# Autodesk Inventor assembly: robot-side-assembly
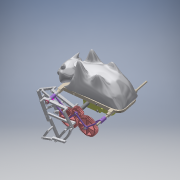
[picture p0: Inventor's stored thumbnail of the model, 180x180]
Saved by Autodesk Inventor 2017 (Build 210142000, 142)
## iProperties
Created: 2021-01-24
Part Number: robot-side-assembly
Document SubType Name: Assembly
Designer: agustin
Author: agustin
## Documents named in this file (42)
- D:\Agustin\Mis proyectos\Mechanisms\WalkingRobot\robot-side-assembly.iam
- D:\Agustin\Mis proyectos\Mechanisms\WalkingRobot\base-bone.ipt
- D:\Agustin\Mis proyectos\Mechanisms\WalkingRobot\bone0.ipt
- D:\Agustin\Mis proyectos\Mechanisms\WalkingRobot\bone1.ipt
- D:\Agustin\Mis proyectos\Mechanisms\WalkingRobot\bone2.ipt
- D:\Agustin\Mis proyectos\Mechanisms\WalkingRobot\bone3.ipt
- D:\Agustin\Mis proyectos\Mechanisms\WalkingRobot\bone4.ipt
- D:\Agustin\Mis proyectos\Mechanisms\WalkingRobot\bone5.ipt
- D:\Agustin\Mis proyectos\Mechanisms\WalkingRobot\toe1.ipt
- D:\Agustin\Mis proyectos\Mechanisms\WalkingRobot\toe2.ipt
- D:\Agustin\Mis proyectos\Mechanisms\WalkingRobot\bone6.ipt
- D:\Agustin\Mis proyectos\Mechanisms\WalkingRobot\bone7.ipt
- D:\Agustin\Mis proyectos\Mechanisms\WalkingRobot\chasis.ipt
- D:\Agustin\Mis proyectos\Mechanisms\WalkingRobot\DCMotor.ipt
- D:\Agustin\Mis proyectos\Mechanisms\WalkingRobot\battery-holder-robot.ipt
- D:\Agustin\Mis proyectos\Mechanisms\WalkingRobot\batter-holder.ipt
- D:\Agustin\Mis proyectos\Mechanisms\WalkingRobot\Servo.ipt
- D:\Agustin\Mis proyectos\Mechanisms\WalkingRobot\base-bone_MIR.ipt
- D:\Agustin\Mis proyectos\Mechanisms\WalkingRobot\bone0_MIR.ipt
- D:\Agustin\Mis proyectos\Mechanisms\WalkingRobot\bone1_MIR.ipt
- D:\Agustin\Mis proyectos\Mechanisms\WalkingRobot\bone2_MIR.ipt
- D:\Agustin\Mis proyectos\Mechanisms\WalkingRobot\bone3_MIR.ipt
- D:\Agustin\Mis proyectos\Mechanisms\WalkingRobot\bone4_MIR.ipt
- D:\Agustin\Mis proyectos\Mechanisms\WalkingRobot\bone5_MIR.ipt
- D:\Agustin\Mis proyectos\Mechanisms\WalkingRobot\toe1_MIR.ipt
- D:\Agustin\Mis proyectos\Mechanisms\WalkingRobot\toe2_MIR.ipt
- D:\Agustin\Mis proyectos\Mechanisms\WalkingRobot\bone6_MIR.ipt
- D:\Agustin\Mis proyectos\Mechanisms\WalkingRobot\bone7_MIR.ipt
- D:\Agustin\Mis proyectos\Mechanisms\WalkingRobot\gear1-shaft.ipt
- D:\Agustin\Mis proyectos\Mechanisms\WalkingRobot\gear-holder.ipt
- D:\Agustin\Mis proyectos\Mechanisms\WalkingRobot\small-gear.ipt
- D:\Agustin\Mis proyectos\Mechanisms\WalkingRobot\big-gear.ipt
- D:\Agustin\Mis proyectos\Mechanisms\WalkingRobot\gear2-shaft.ipt
- D:\Agustin\Mis proyectos\Mechanisms\WalkingRobot\dc-driver.ipt
- D:\Agustin\Mis proyectos\Mechanisms\WalkingRobot\node-mcu.ipt
- D:\Agustin\Mis proyectos\Mechanisms\WalkingRobot\ultrasound.ipt
- D:\Agustin\Mis proyectos\Mechanisms\WalkingRobot\head.ipt
- D:\Agustin\Mis proyectos\Mechanisms\WalkingRobot\shell.ipt
- D:\Agustin\Mis proyectos\Mechanisms\WalkingRobot\servo-shaft.ipt
- C:\Users\agustin\Documents\Inventor\Content Center Files\R2017\en-US\ANSI B18.3.4M(2)\ANSI B18.3.4M - M3 x 0.5 x 25(1).ipt
- C:\Users\agustin\Documents\Inventor\Content Center Files\R2017\en-US\AS 1112 (4)\AS 1112 - M3(2).ipt
- D:\Agustin\Mis proyectos\Mechanisms\WalkingRobot\washer.ipt
## Components (51 placed, 41 different names)
1. base-bone:1 — Mate:1, Mate:2, Mate:3, Mate:5, Mate:13, Mate:15, Mate:17, Mate:18
2. bone0:1 — Mate:5, Mate:6, Mate:22, Mate:25, Mate:152, Mate:154, Mate:194
3. bone1:1 — Mate:3, Mate:4, Mate:11, Mate:17, Mate:19, Mate:20
4. bone2:1 — Mate:2, Mate:12, Mate:18
5. bone3:1 — Mate:10, Mate:11, Mate:12, Mate:20
6. bone4:1 — Mate:4, Mate:7, Mate:8, Mate:19, Mate:23
7. bone5:1 — Mate:6, Mate:7, Mate:14, Mate:21, Mate:22
8. toe1:1 — Mate:8, Mate:9, Mate:23, Mate:24
9. toe2:1 — Mate:9, Mate:10, Mate:24
10. bone6:1 — Mate:1, Mate:16, Mate:153, Angle:3, Mate:156
11. bone7:1 — Mate:13, Mate:14, Mate:15, Mate:16, Mate:21
12. chasis:1 — Mate:25, Mate:121, Mate:122, Mate:134, Mate:152, Angle:6, Angle:7, Angle:8, Mate:166, Mate:167, Mate:168, Mate:169, Mate:172, Mate:173, Mate:174, Mate:175, Mate:176, Mate:177, Mate:178, Angle:11, Flush:13, Flush:14, Mate:189, Mate:190, Mate:191, Angle:12, Mate:193
13. battery-holder-robot:1 — Mate:44, Mate:179, Mate:180, Angle:11, Flush:11, Flush:12, Mate:192
14. batter-holder:1 — Mate:44, Mate:192
15. Servo:1 — Mate:163, Mate:164, Mate:191, Angle:12
16. base-bone_MIR:1 — Mate:49, Mate:50, Mate:51, Mate:52, Mate:53, Mate:67, Mate:70, Mate:72
17. bone0_MIR:1 — Mate:49, Mate:59, Mate:61, Mate:121, Mate:122
18. bone1_MIR:1 — Mate:50, Mate:51, Mate:54, Mate:56, Mate:57, Mate:58
19. bone2_MIR:1 — Mate:52, Mate:53, Mate:55
20. bone3_MIR:1 — Mate:54, Mate:55, Mate:56, Mate:65
21. bone4_MIR:1 — Mate:57, Mate:58, Mate:60, Mate:62, Mate:63
22. bone5_MIR:1 — Mate:59, Mate:60, Mate:61, Mate:68, Mate:71
23. toe1_MIR:1 — Mate:62, Mate:63, Mate:64, Mate:66
24. toe2_MIR:1 — Mate:64, Mate:65, Mate:66
25. bone6_MIR:1 — Mate:67, Mate:69, Mate:146, Angle:3
26. bone7_MIR:1 — Mate:68, Mate:69, Mate:70, Mate:71, Mate:72
27. gear1-shaft:1 — Mate:135, Mate:138, Mate:151, Angle:5, Mate:170, Mate:171
28. gear-holder:1 — Mate:134, Mate:135, Mate:136, Mate:137, Mate:144, Mate:146, Mate:147, Mate:151
29. gear-holder:2 — Mate:136, Mate:137, Mate:139, Mate:140, Mate:147, Mate:153, Mate:154
30. Spur Gear2:1 — Mate:138, Flush:5, Flush:6, Mate:144, Rotation:1, Angle:5, Rotation:2
31. Spur Gear1:1 — Mate:139, Flush:6, Mate:142, Flush:8, Mate:155, Rotation:1
32. Spur Gear1:2 — Mate:140, Flush:5, Mate:141, Mate:143, Flush:7, Rotation:2
33. gear2-shaft:1 — Mate:141, Mate:143, Flush:7
34. gear2-shaft:2 — Mate:142, Flush:8, Mate:155, Mate:156
35. dc-driver:1 — Angle:6, Angle:9, Mate:189
36. node-mcu:1 — Angle:7, Angle:8, Angle:9, Mate:190
37. ultrasound:1 — Mate:161, Mate:162, Angle:10
38. head:1 — Mate:161, Mate:162, Angle:10, Mate:165, Flush:9, Flush:10
39. shell:1 — Mate:166
40. servo-shaft:1 — Mate:163, Mate:164, Mate:165, Flush:9, Flush:10
41. DCMotor:1 — Mate:167, Mate:168, Mate:169, Mate:170, Mate:171, Mate:181, Mate:182
42. DCMotor:2 — Mate:172, Mate:173, Mate:174, Mate:179, Mate:180, Mate:183, Mate:184
43. Forged Hexagon Socket Button Head Cap Screw - Metric M3 x 0.5 x 25:1 — Mate:176, Mate:177, Mate:188
44. Forged Hexagon Socket Button Head Cap Screw - Metric M3 x 0.5 x 25:2 — Mate:175, Mate:178, Mate:187
45. Forged Hexagon Socket Button Head Cap Screw - Metric M3 x 0.5 x 25:3 — Mate:181, Mate:182, Mate:186
46. Forged Hexagon Socket Button Head Cap Screw - Metric M3 x 0.5 x 25:4 — Mate:183, Mate:184, Mate:185
47. AS 1112 (4) - Metric M3:1 — Mate:185, Flush:12
48. AS 1112 (4) - Metric M3:2 — Mate:187, Flush:13
49. AS 1112 (4) - Metric M3:3 — Mate:188, Flush:14
50. AS 1112 (4) - Metric M3:4 — Mate:186, Flush:11
51. washer:1 — Mate:193, Mate:194
## Relationships (126: Mate 105, Flush 10, Angle 9, RelateRotation 2)
- Mate:1: base-bone:1 ↔ bone6:1
- Mate:2: base-bone:1 ↔ bone2:1
- Mate:3: base-bone:1 ↔ bone1:1
- Mate:4: bone1:1 ↔ bone4:1
- Mate:5: base-bone:1 ↔ bone0:1
- Mate:6: bone0:1 ↔ bone5:1
- Mate:7: bone4:1 ↔ bone5:1
- Mate:8: bone4:1 ↔ toe1:1
- Mate:9: toe1:1 ↔ toe2:1
- Mate:10: bone3:1 ↔ toe2:1
- Mate:11: bone1:1 ↔ bone3:1
- Mate:12: bone2:1 ↔ bone3:1
- Mate:13: base-bone:1 ↔ bone7:1
- Mate:14: bone5:1 ↔ bone7:1
- Mate:15: base-bone:1 ↔ bone7:1
- Mate:16: bone6:1 ↔ bone7:1
- Mate:17: base-bone:1 ↔ bone1:1
- Mate:18: base-bone:1 ↔ bone2:1
- Mate:19: bone1:1 ↔ bone4:1
- Mate:20: bone1:1 ↔ bone3:1
- Mate:21: bone5:1 ↔ bone7:1
- Mate:22: bone0:1 ↔ bone5:1
- Mate:23: bone4:1 ↔ toe1:1
- Mate:24: toe1:1 ↔ toe2:1
- Mate:25: bone0:1 ↔ chasis:1
- Mate:44: battery-holder-robot:1 ↔ batter-holder:1
- Mate:49: base-bone_MIR:1 ↔ bone0_MIR:1
- Mate:50: base-bone_MIR:1 ↔ bone1_MIR:1
- Mate:51: base-bone_MIR:1 ↔ bone1_MIR:1
- Mate:52: base-bone_MIR:1 ↔ bone2_MIR:1
- Mate:53: base-bone_MIR:1 ↔ bone2_MIR:1
- Mate:54: bone1_MIR:1 ↔ bone3_MIR:1
- Mate:55: bone2_MIR:1 ↔ bone3_MIR:1
- Mate:56: bone1_MIR:1 ↔ bone3_MIR:1
- Mate:57: bone1_MIR:1 ↔ bone4_MIR:1
- Mate:58: bone1_MIR:1 ↔ bone4_MIR:1
- Mate:59: bone0_MIR:1 ↔ bone5_MIR:1
- Mate:60: bone4_MIR:1 ↔ bone5_MIR:1
- Mate:61: bone0_MIR:1 ↔ bone5_MIR:1
- Mate:62: bone4_MIR:1 ↔ toe1_MIR:1
- Mate:63: bone4_MIR:1 ↔ toe1_MIR:1
- Mate:64: toe1_MIR:1 ↔ toe2_MIR:1
- Mate:65: bone3_MIR:1 ↔ toe2_MIR:1
- Mate:66: toe1_MIR:1 ↔ toe2_MIR:1
- Mate:67: base-bone_MIR:1 ↔ bone6_MIR:1
- Mate:68: bone5_MIR:1 ↔ bone7_MIR:1
- Mate:69: bone6_MIR:1 ↔ bone7_MIR:1
- Mate:70: base-bone_MIR:1 ↔ bone7_MIR:1
- Mate:71: bone5_MIR:1 ↔ bone7_MIR:1
- Mate:72: base-bone_MIR:1 ↔ bone7_MIR:1
- Mate:121: chasis:1 ↔ bone0_MIR:1
- Mate:122: chasis:1 ↔ bone0_MIR:1
- Mate:134: chasis:1 ↔ gear-holder:1
- Mate:135: gear1-shaft:1 ↔ gear-holder:1
- Mate:136: gear-holder:1 ↔ gear-holder:2
- Mate:137: gear-holder:1 ↔ gear-holder:2
- Mate:138: gear1-shaft:1 ↔ Spur Gear2:1
- Mate:139: gear-holder:2 ↔ Spur Gear1:1
- Mate:140: gear-holder:2 ↔ Spur Gear1:2
- Flush:5: Spur Gear2:1 ↔ Spur Gear1:2
- Flush:6: Spur Gear2:1 ↔ Spur Gear1:1
- Mate:141: Spur Gear1:2 ↔ gear2-shaft:1
- Mate:142: Spur Gear1:1 ↔ gear2-shaft:2
- Mate:143: Spur Gear1:2 ↔ gear2-shaft:1
- Mate:144: gear-holder:1 ↔ Spur Gear2:1
- Mate:146: bone6_MIR:1 ↔ gear-holder:1
- Flush:7: Spur Gear1:2 ↔ gear2-shaft:1
- Flush:8: Spur Gear1:1 ↔ gear2-shaft:2
- Mate:147: gear-holder:1 ↔ gear-holder:2
- Mate:151: gear1-shaft:1 ↔ gear-holder:1
- Mate:152: bone0:1 ↔ chasis:1
- Mate:153: bone6:1 ↔ gear-holder:2
- Mate:154: bone0:1 ↔ gear-holder:2
- Angle:3 (0 deg): bone6:1 ↔ bone6_MIR:1
- Mate:155: Spur Gear1:1 ↔ gear2-shaft:2
- Mate:156: bone6:1 ↔ gear2-shaft:2
- Rotation:1 [RelateRotation] (1.9565 ul): Spur Gear2:1 ↔ Spur Gear1:1
- Angle:5 (0 deg): gear1-shaft:1 ↔ Spur Gear2:1
- Rotation:2 [RelateRotation] (1.9565 ul): Spur Gear2:1 ↔ Spur Gear1:2
- Angle:6 (0 deg): chasis:1 ↔ dc-driver:1
- Angle:7 (0 deg): chasis:1 ↔ node-mcu:1
- Angle:8 (0 deg): chasis:1 ↔ node-mcu:1
- Angle:9 (0 deg): dc-driver:1 ↔ node-mcu:1
- Mate:161: ultrasound:1 ↔ head:1
- Mate:162: ultrasound:1 ↔ head:1
- Angle:10 (180 deg): ultrasound:1 ↔ head:1
- Mate:163: Servo:1 ↔ servo-shaft:1
- Mate:164: Servo:1 ↔ servo-shaft:1
- Mate:165: head:1 ↔ servo-shaft:1
- Flush:9: head:1 ↔ servo-shaft:1
- Flush:10: head:1 ↔ servo-shaft:1
- Mate:166: chasis:1 ↔ shell:1
- Mate:167: chasis:1 ↔ DCMotor:1
- Mate:168: chasis:1 ↔ DCMotor:1
- Mate:169: chasis:1 ↔ DCMotor:1
- Mate:170: gear1-shaft:1 ↔ DCMotor:1
- Mate:171: gear1-shaft:1 ↔ DCMotor:1
- Mate:172: chasis:1 ↔ DCMotor:2
- Mate:173: chasis:1 ↔ DCMotor:2
- Mate:174: chasis:1 ↔ DCMotor:2
- Mate:175: chasis:1 ↔ Forged Hexagon Socket Button Head Cap Screw - Metric M3 x 0.5 x 25:2
- Mate:176: chasis:1 ↔ Forged Hexagon Socket Button Head Cap Screw - Metric M3 x 0.5 x 25:1
- Mate:177: chasis:1 ↔ Forged Hexagon Socket Button Head Cap Screw - Metric M3 x 0.5 x 25:1
- Mate:178: chasis:1 ↔ Forged Hexagon Socket Button Head Cap Screw - Metric M3 x 0.5 x 25:2
- Mate:179: battery-holder-robot:1 ↔ DCMotor:2
- Mate:180: battery-holder-robot:1 ↔ DCMotor:2
- Angle:11 (0 deg): chasis:1 ↔ battery-holder-robot:1
- Mate:181: DCMotor:1 ↔ Forged Hexagon Socket Button Head Cap Screw - Metric M3 x 0.5 x 25:3
- Mate:182: DCMotor:1 ↔ Forged Hexagon Socket Button Head Cap Screw - Metric M3 x 0.5 x 25:3
- Mate:183: DCMotor:2 ↔ Forged Hexagon Socket Button Head Cap Screw - Metric M3 x 0.5 x 25:4
- Mate:184: DCMotor:2 ↔ Forged Hexagon Socket Button Head Cap Screw - Metric M3 x 0.5 x 25:4
- Mate:185: Forged Hexagon Socket Button Head Cap Screw - Metric M3 x 0.5 x 25:4 ↔ AS 1112 (4) - Metric M3:1
- Mate:186: Forged Hexagon Socket Button Head Cap Screw - Metric M3 x 0.5 x 25:3 ↔ AS 1112 (4) - Metric M3:4
- Mate:187: Forged Hexagon Socket Button Head Cap Screw - Metric M3 x 0.5 x 25:2 ↔ AS 1112 (4) - Metric M3:2
- Mate:188: Forged Hexagon Socket Button Head Cap Screw - Metric M3 x 0.5 x 25:1 ↔ AS 1112 (4) - Metric M3:3
- Flush:11: battery-holder-robot:1 ↔ AS 1112 (4) - Metric M3:4
- Flush:12: battery-holder-robot:1 ↔ AS 1112 (4) - Metric M3:1
- Flush:13: chasis:1 ↔ AS 1112 (4) - Metric M3:2
- Flush:14: chasis:1 ↔ AS 1112 (4) - Metric M3:3
- Mate:189: chasis:1 ↔ dc-driver:1
- Mate:190: chasis:1 ↔ node-mcu:1
- Mate:191: chasis:1 ↔ Servo:1
- Angle:12 (0 deg): chasis:1 ↔ Servo:1
- Mate:192: battery-holder-robot:1 ↔ batter-holder:1
- Mate:193: chasis:1 ↔ washer:1
- Mate:194: bone0:1 ↔ washer:1
